# Autodesk Inventor assembly: FAN CONSTRAINED
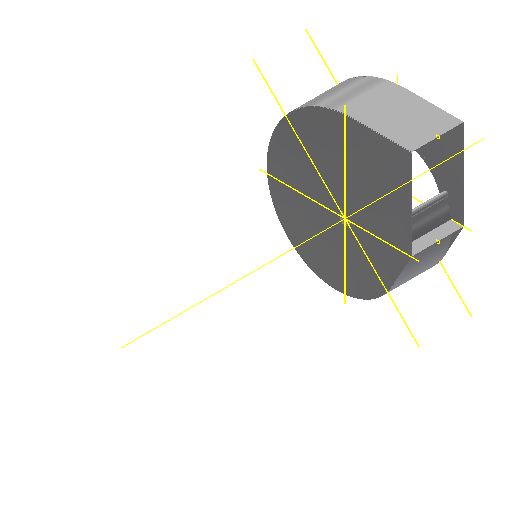
[picture p0: Inventor's stored thumbnail of the model, 512x512]
Saved by Autodesk Inventor 2022 (Build 260148000, 148)
## iProperties
Created: 2007-05-11
Part Number: FAN CONSTRAINED
Document SubType Name: Assembly
Designer: LionelF
Mass: 99948.8 g
Surface Area: 80653.8 cm^2
Volume: 12716.1 cm^3
Density: 7.86 g/cm^3
Author: LionelF
## Documents named in this file (6)
- D:\Autodesk Inventor 2021 Advanced Assembly Modeling Practice Files\Blower\FAN CONSTRAINED.iam
- D:\Autodesk Inventor 2021 Advanced Assembly Modeling Practice Files\Blower\drive side sheet.ipt
- D:\Autodesk Inventor 2021 Advanced Assembly Modeling Practice Files\Blower\band.ipt
- D:\Autodesk Inventor 2021 Advanced Assembly Modeling Practice Files\Blower\inlet side sheet.ipt
- D:\Autodesk Inventor 2021 Advanced Assembly Modeling Practice Files\Blower\cutoff pipe.ipt
- D:\Autodesk Inventor 2021 Advanced Assembly Modeling Practice Files\Blower\outlet strip.ipt
## Components (5 placed, 5 different names)
1. drive side sheet:1 — Mate:1, Mate:2, Mate:5, Mate:6, Flush:1, Mate:8, Mate:10
2. band:2 — Mate:1, Mate:2, Mate:3, Mate:4, Tangent:1, Tangent:2
3. inlet side sheet:1 — Mate:3, Mate:4, Mate:5, Mate:6, Flush:1, Mate:9
4. cutoff pipe:1 — Mate:10, Tangent:1, Tangent:2
5. outlet strip:1 — Mate:8, Mate:9
## Relationships (13: Mate 10, Tangent 2, Flush 1)
- Mate:1: drive side sheet:1 ↔ band:2
- Mate:2: drive side sheet:1 ↔ band:2
- Mate:3: band:2 ↔ inlet side sheet:1
- Mate:4: band:2 ↔ inlet side sheet:1
- Mate:5: drive side sheet:1 ↔ inlet side sheet:1
- Mate:6: drive side sheet:1 ↔ inlet side sheet:1
- Flush:1: drive side sheet:1 ↔ inlet side sheet:1
- [Mate]: drive side sheet:1 ↔ outlet strip:1
- Mate:8: drive side sheet:1 ↔ outlet strip:1
- Mate:9: inlet side sheet:1 ↔ outlet strip:1
- Mate:10: drive side sheet:1 ↔ cutoff pipe:1
- Tangent:1: band:2 ↔ cutoff pipe:1
- Tangent:2: band:2 ↔ cutoff pipe:1
